# Autodesk Inventor assembly: Holder_21700_Dual
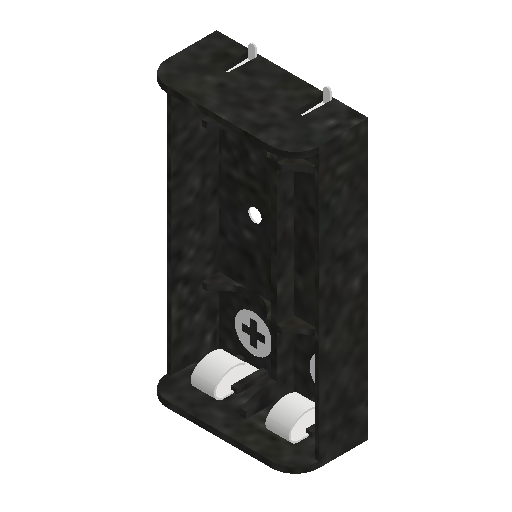
[picture p0: Inventor's stored thumbnail of the model, 512x512]
Saved by Autodesk Inventor 2025.2 (Build 292293000, 293)
## iProperties
Created: 2025-03-09
Part Number: Holder_21700_Dual
Document SubType Name: Assembly
Designer: ahorat
Author: ahorat
## Documents named in this file (3)
- C:\Daten\Temp\R32EntrySystem\cad\UPS_HAT_E\Holder_21700_Dual.iam
- C:\Daten\Temp\R32EntrySystem\cad\UPS_HAT_E\Holder_21700_Dual.ipt
- C:\Daten\Temp\R32EntrySystem\cad\UPS_HAT_E\Holder_Metal.ipt
## Components (5 placed, 2 different names)
1. Holder_21700_Dual:1 — Mate:1, Mate:2, Mate:3, Mate:4, Mate:5, Mate:6, Mate:7, Mate:8, Mate:9, Mate:10, Mate:11, Mate:12
2. Holder_Metal:1 — Mate:1, Mate:2, Mate:3
3. Holder_Metal:2 — Mate:4, Mate:5, Mate:6
4. Holder_Metal:3 — Mate:7, Mate:10, Mate:11
5. Holder_Metal:4 — Mate:8, Mate:9, Mate:12
## Relationships (12: Mate 12)
- Mate:1: Holder_21700_Dual:1 ↔ Holder_Metal:1
- Mate:2: Holder_21700_Dual:1 ↔ Holder_Metal:1
- Mate:3: Holder_21700_Dual:1 ↔ Holder_Metal:1
- Mate:4: Holder_21700_Dual:1 ↔ Holder_Metal:2
- Mate:5: Holder_21700_Dual:1 ↔ Holder_Metal:2
- Mate:6: Holder_21700_Dual:1 ↔ Holder_Metal:2
- Mate:7: Holder_21700_Dual:1 ↔ Holder_Metal:3
- Mate:8: Holder_21700_Dual:1 ↔ Holder_Metal:4
- Mate:9: Holder_21700_Dual:1 ↔ Holder_Metal:4
- Mate:10: Holder_21700_Dual:1 ↔ Holder_Metal:3
- Mate:11: Holder_21700_Dual:1 ↔ Holder_Metal:3
- Mate:12: Holder_21700_Dual:1 ↔ Holder_Metal:4
